# Autodesk Inventor assembly: 110033226_iam_10_角落碉堡
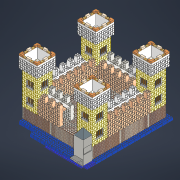
[picture p0: Inventor's stored thumbnail of the model, 180x180]
Saved by Autodesk Inventor 2022 (Build 260153000, 153)
## iProperties
Created: 2022-06-28
Part Number: 110033226_iam_10_角落碉堡
Document SubType Name: Assembly
Designer: User
Author: User
## Documents named in this file (8)
- D:\D-disk\pomelo\大一\下學期\機械設計製圖\1100332260_LEGOproj_沒有公主城堡\110033226_iam_10_角落碉堡.iam
- D:\D-disk\pomelo\大一\下學期\機械設計製圖\1100332260_LEGOproj_沒有公主城堡\110033226_ipt_43_角落碉堡基座.ipt
- D:\D-disk\pomelo\大一\下學期\機械設計製圖\1100332260_LEGOproj_沒有公主城堡\110033226_ipt_04_小河.ipt
- D:\D-disk\pomelo\大一\下學期\機械設計製圖\1100332260_LEGOproj_沒有公主城堡\110033226_iam_06_城堡四角塔.iam
- D:\D-disk\pomelo\大一\下學期\機械設計製圖\1100332260_LEGOproj_沒有公主城堡\110033226_ipt_34_中心城堡圍牆.ipt
- D:\D-disk\pomelo\大一\下學期\機械設計製圖\1100332260_LEGOproj_沒有公主城堡\110033226_ipt_24_直條(3x1).ipt
- D:\D-disk\pomelo\大一\下學期\機械設計製圖\1100332260_LEGOproj_沒有公主城堡\110033226_ipt_46_水中房子.ipt
- D:\D-disk\pomelo\大一\下學期\機械設計製圖\1100332260_LEGOproj_沒有公主城堡\110033226_ipt_37_小河方塊.ipt
## Components (310 placed, 7 different names)
1. 110033226_ipt_34_中心城堡圍牆:39 — 貼合:27, 貼合:28, 貼合:29, 貼合:38
2. 110033226_ipt_46_水中房子:1 — 貼合:39, 貼合:40, 貼合:41, 貼合:45, 貼合:46, 貼合:48, 貼合:50
3. 110033226_ipt_43_角落碉堡基座:1 — 貼合:1, 貼合:2, 貼合:3, 貼合:4, 貼合:5, 貼合:6, 貼合:7, 貼合:8, 貼合:9, 貼合:11, 貼合:39
4. 110033226_ipt_43_角落碉堡基座:2
5. 110033226_ipt_43_角落碉堡基座:3
6. 110033226_ipt_43_角落碉堡基座:4
7. 110033226_ipt_43_角落碉堡基座:5 — 貼合:40
8. 110033226_ipt_43_角落碉堡基座:6
9. 110033226_ipt_43_角落碉堡基座:7
10. 110033226_ipt_43_角落碉堡基座:8
11. 110033226_ipt_43_角落碉堡基座:9
12. 110033226_ipt_43_角落碉堡基座:10
13. 110033226_ipt_43_角落碉堡基座:11
14. 110033226_ipt_43_角落碉堡基座:12
15. 110033226_ipt_43_角落碉堡基座:13
16. 110033226_ipt_43_角落碉堡基座:14
17. 110033226_ipt_43_角落碉堡基座:15 — 貼合:12, 貼合:13, 貼合:14, 貼合:15, 貼合:16, 貼合:17, 貼合:18, 貼合:19, 貼合:21, 貼合:22, 貼合:23, 貼合:24, 貼合:25, 貼合:26, 貼合:27, 貼合:28, 貼合:29, 貼合:30, 貼合:31, 貼合:32, 貼合:33, 貼合:34, 貼合:35, 貼合:36, 貼合:37
18. 110033226_ipt_04_小河:4 — 貼合:7, 貼合:8, 貼合:9, 貼合:41, 貼合:42, 貼合:43, 貼合:44
19. 110033226_ipt_04_小河:5
20. 110033226_ipt_04_小河:6
21. 110033226_ipt_04_小河:7
22. 110033226_ipt_04_小河:8
23. 110033226_ipt_04_小河:9
24. 110033226_ipt_04_小河:10
25. 110033226_ipt_04_小河:11
26. 110033226_ipt_04_小河:12
27. 110033226_ipt_04_小河:13
28. 110033226_ipt_04_小河:14
29. 110033226_ipt_04_小河:15
30. 110033226_ipt_04_小河:16
31. 110033226_ipt_04_小河:17
32. 110033226_ipt_04_小河:18
33. 110033226_ipt_04_小河:19
34. 110033226_ipt_04_小河:20
35. 110033226_ipt_04_小河:21
36. 110033226_ipt_04_小河:22
37. 110033226_ipt_04_小河:23
38. 110033226_ipt_04_小河:24
39. 110033226_ipt_04_小河:25
40. 110033226_ipt_04_小河:26
41. 110033226_ipt_04_小河:27
42. 110033226_ipt_04_小河:28
43. 110033226_ipt_04_小河:29
44. 110033226_ipt_04_小河:30
45. 110033226_ipt_04_小河:31
46. 110033226_ipt_04_小河:32
47. 110033226_ipt_04_小河:33
48. 110033226_ipt_04_小河:34
49. 110033226_ipt_04_小河:35
50. 110033226_ipt_04_小河:36
51. 110033226_ipt_04_小河:37
52. 110033226_ipt_04_小河:38
53. 110033226_ipt_04_小河:39
54. 110033226_ipt_04_小河:40
55. 110033226_ipt_04_小河:41
56. 110033226_ipt_04_小河:42
57. 110033226_ipt_04_小河:43 — 對稱:1, 貼合:10
58. 110033226_ipt_04_小河:44
59. 110033226_ipt_04_小河:45
60. 110033226_ipt_04_小河:3 — 對稱:1, 貼合:10, 貼合:11
61. 110033226_ipt_04_小河:46
62. 110033226_ipt_04_小河:47
63. 110033226_ipt_04_小河:48
64. 110033226_ipt_04_小河:49
65. 110033226_ipt_04_小河:50
66. 110033226_ipt_04_小河:51
67. 110033226_ipt_04_小河:52
68. 110033226_ipt_04_小河:53
69. 110033226_ipt_04_小河:54
70. 110033226_ipt_04_小河:55
71. 110033226_ipt_04_小河:56
72. 110033226_ipt_04_小河:57
73. 110033226_ipt_04_小河:58
74. 110033226_ipt_04_小河:59
75. 110033226_ipt_04_小河:60
76. 110033226_ipt_04_小河:61
77. 110033226_ipt_04_小河:62
78. 110033226_ipt_04_小河:63
79. 110033226_ipt_04_小河:64
80. 110033226_ipt_04_小河:65
81. 110033226_ipt_04_小河:66
82. 110033226_ipt_04_小河:67
83. 110033226_ipt_04_小河:68
84. 110033226_ipt_04_小河:69
85. 110033226_ipt_04_小河:70
86. 110033226_ipt_04_小河:71
87. 110033226_ipt_04_小河:72
88. 110033226_ipt_04_小河:73
89. 110033226_ipt_04_小河:74
90. 110033226_ipt_04_小河:75
91. 110033226_ipt_04_小河:76
92. 110033226_ipt_04_小河:77
93. 110033226_ipt_04_小河:78
94. 110033226_ipt_04_小河:79
95. 110033226_ipt_04_小河:80
96. 110033226_ipt_04_小河:81
97. 110033226_ipt_04_小河:82
98. 110033226_ipt_04_小河:83
99. 110033226_iam_06_城堡四角塔:1 [sub-assembly] — 貼合:12, 貼合:13, 貼合:14
100. 110033226_iam_06_城堡四角塔:2 [sub-assembly]
101. 110033226_iam_06_城堡四角塔:3 [sub-assembly]
102. 110033226_iam_06_城堡四角塔:4 [sub-assembly]
103. 110033226_ipt_34_中心城堡圍牆:3 — 貼合:18, 貼合:19, 貼合:20
104. 110033226_ipt_34_中心城堡圍牆:1 — 貼合:15, 貼合:16, 貼合:17, 貼合:20
105. 110033226_ipt_34_中心城堡圍牆:5
106. 110033226_ipt_34_中心城堡圍牆:6
107. 110033226_ipt_34_中心城堡圍牆:7
108. 110033226_ipt_34_中心城堡圍牆:8
109. 110033226_ipt_34_中心城堡圍牆:9
110. 110033226_ipt_34_中心城堡圍牆:10
111. 110033226_ipt_34_中心城堡圍牆:11
112. 110033226_ipt_34_中心城堡圍牆:12
113. 110033226_ipt_34_中心城堡圍牆:13
114. 110033226_ipt_34_中心城堡圍牆:14
115. 110033226_ipt_34_中心城堡圍牆:15
116. 110033226_ipt_34_中心城堡圍牆:16
117. 110033226_ipt_34_中心城堡圍牆:17
118. 110033226_ipt_34_中心城堡圍牆:18
119. 110033226_ipt_34_中心城堡圍牆:19
120. 110033226_ipt_34_中心城堡圍牆:20
121. 110033226_ipt_34_中心城堡圍牆:21
122. 110033226_ipt_34_中心城堡圍牆:22
123. 110033226_ipt_34_中心城堡圍牆:23
124. 110033226_ipt_34_中心城堡圍牆:24
125. 110033226_ipt_34_中心城堡圍牆:25
126. 110033226_ipt_34_中心城堡圍牆:26
127. 110033226_ipt_34_中心城堡圍牆:28 — 貼合:25, 齊平:1, 貼合:26
128. 110033226_ipt_34_中心城堡圍牆:27 — 貼合:21, 貼合:22, 貼合:23, 貼合:24, 齊平:1
129. 110033226_ipt_34_中心城堡圍牆:29
130. 110033226_ipt_34_中心城堡圍牆:30
131. 110033226_ipt_34_中心城堡圍牆:31
132. 110033226_ipt_34_中心城堡圍牆:32
133. 110033226_ipt_34_中心城堡圍牆:33
134. 110033226_ipt_34_中心城堡圍牆:34
135. 110033226_ipt_34_中心城堡圍牆:35
136. 110033226_ipt_34_中心城堡圍牆:36
137. 110033226_ipt_34_中心城堡圍牆:37
138. 110033226_ipt_34_中心城堡圍牆:38
139. 110033226_ipt_34_中心城堡圍牆:41 — 貼合:33, 貼合:34, 貼合:35
140. 110033226_ipt_34_中心城堡圍牆:40 — 貼合:30, 貼合:31, 貼合:32
141. 110033226_ipt_34_中心城堡圍牆:42
142. 110033226_ipt_34_中心城堡圍牆:43
143. 110033226_ipt_37_小河方塊:21 — 貼合:45, 貼合:46, 貼合:47
144. 110033226_ipt_37_小河方塊:22
145. 110033226_ipt_37_小河方塊:23
146. 110033226_ipt_37_小河方塊:24
147. 110033226_ipt_37_小河方塊:25
148. 110033226_ipt_37_小河方塊:26 — 貼合:49
149. 110033226_ipt_37_小河方塊:27
150. 110033226_ipt_37_小河方塊:28
151. 110033226_ipt_37_小河方塊:29
152. 110033226_ipt_37_小河方塊:30
153. 110033226_ipt_37_小河方塊:31
154. 110033226_ipt_37_小河方塊:32
155. 110033226_ipt_37_小河方塊:33
156. 110033226_ipt_37_小河方塊:34
157. 110033226_ipt_37_小河方塊:35
158. 110033226_ipt_37_小河方塊:36
159. 110033226_ipt_37_小河方塊:37
160. 110033226_ipt_37_小河方塊:38
161. 110033226_ipt_37_小河方塊:39
162. 110033226_ipt_37_小河方塊:40
163. 110033226_ipt_24_直條(3x1):1 — 貼合:36, 貼合:37, 貼合:38
164. 110033226_ipt_24_直條(3x1):2
165. 110033226_ipt_24_直條(3x1):3
166. 110033226_ipt_24_直條(3x1):4
167. 110033226_ipt_24_直條(3x1):5
168. 110033226_ipt_24_直條(3x1):6
169. 110033226_ipt_24_直條(3x1):7
170. 110033226_ipt_24_直條(3x1):8
171. 110033226_ipt_24_直條(3x1):9
172. 110033226_ipt_24_直條(3x1):10
173. 110033226_ipt_24_直條(3x1):11
174. 110033226_ipt_24_直條(3x1):12
175. 110033226_ipt_37_小河方塊:1 — 貼合:42, 貼合:43, 貼合:44
176. 110033226_ipt_37_小河方塊:2
177. 110033226_ipt_37_小河方塊:3
178. 110033226_ipt_37_小河方塊:4
179. 110033226_ipt_37_小河方塊:5
180. 110033226_ipt_37_小河方塊:6
181. 110033226_ipt_37_小河方塊:7
182. 110033226_ipt_37_小河方塊:8
183. 110033226_ipt_37_小河方塊:9
184. 110033226_ipt_37_小河方塊:10 — 貼合:47
185. 110033226_ipt_37_小河方塊:11
186. 110033226_ipt_37_小河方塊:12
187. 110033226_ipt_37_小河方塊:13
188. 110033226_ipt_37_小河方塊:14
189. 110033226_ipt_37_小河方塊:15
190. 110033226_ipt_37_小河方塊:16
191. 110033226_ipt_37_小河方塊:17
192. 110033226_ipt_37_小河方塊:18
193. 110033226_ipt_37_小河方塊:19
194. 110033226_ipt_37_小河方塊:20
195. 110033226_ipt_04_小河:88 — 貼合:48, 貼合:49, 貼合:50
196. 110033226_ipt_04_小河:89
197. 110033226_ipt_04_小河:90
198. 110033226_ipt_04_小河:91
199. 110033226_ipt_04_小河:92
200. 110033226_ipt_04_小河:93
201. 110033226_ipt_04_小河:94
202. 110033226_ipt_04_小河:95
203. 110033226_ipt_04_小河:96
204. 110033226_ipt_04_小河:97
205. 110033226_ipt_04_小河:98
206. 110033226_ipt_04_小河:99
207. 110033226_ipt_04_小河:100
208. 110033226_ipt_04_小河:101
209. 110033226_ipt_04_小河:102
210. 110033226_ipt_04_小河:103
211. 110033226_ipt_04_小河:104
212. 110033226_ipt_04_小河:105
213. 110033226_ipt_04_小河:106
214. 110033226_ipt_04_小河:107
215. 110033226_ipt_04_小河:108
216. 110033226_ipt_04_小河:109
217. 110033226_ipt_04_小河:110
218. 110033226_ipt_04_小河:111
219. 110033226_ipt_04_小河:1 — 貼合:4, 貼合:5, 貼合:6
220. 110033226_ipt_04_小河:84
221. 110033226_ipt_04_小河:85
222. 110033226_ipt_04_小河:86
223. 110033226_ipt_04_小河:87
224. 110033226_ipt_04_小河:112
225. 110033226_ipt_04_小河:113
226. 110033226_ipt_04_小河:114
227. 110033226_ipt_04_小河:115
228. 110033226_ipt_04_小河:116
229. 110033226_ipt_04_小河:117
230. 110033226_ipt_04_小河:118
231. 110033226_ipt_04_小河:119
232. 110033226_ipt_04_小河:120
233. 110033226_ipt_04_小河:121
234. 110033226_ipt_04_小河:122
235. 110033226_ipt_04_小河:123
236. 110033226_ipt_04_小河:124
237. 110033226_ipt_04_小河:125
238. 110033226_ipt_04_小河:126
239. 110033226_ipt_04_小河:127
240. 110033226_ipt_04_小河:128
241. 110033226_ipt_04_小河:129
242. 110033226_ipt_04_小河:130
243. 110033226_ipt_04_小河:131
244. 110033226_ipt_04_小河:132
245. 110033226_ipt_04_小河:133
246. 110033226_ipt_04_小河:134
247. 110033226_ipt_04_小河:135
248. 110033226_ipt_04_小河:136
249. 110033226_ipt_04_小河:137
250. 110033226_ipt_04_小河:138
251. 110033226_ipt_04_小河:139
252. 110033226_ipt_04_小河:140
253. 110033226_ipt_04_小河:141
254. 110033226_ipt_04_小河:142
255. 110033226_ipt_04_小河:143
256. 110033226_ipt_04_小河:144
257. 110033226_ipt_04_小河:145
258. 110033226_ipt_04_小河:146
259. 110033226_ipt_04_小河:147
260. 110033226_ipt_04_小河:148
261. 110033226_ipt_04_小河:149
262. 110033226_ipt_04_小河:150
263. 110033226_ipt_04_小河:151
264. 110033226_ipt_04_小河:152
265. 110033226_ipt_04_小河:153
266. 110033226_ipt_04_小河:154
267. 110033226_ipt_04_小河:155
268. 110033226_ipt_04_小河:156
269. 110033226_ipt_04_小河:157
270. 110033226_ipt_04_小河:158
271. 110033226_ipt_04_小河:159
272. 110033226_ipt_04_小河:160
273. 110033226_ipt_04_小河:161
274. 110033226_ipt_04_小河:162
275. 110033226_ipt_04_小河:163
276. 110033226_ipt_04_小河:164
277. 110033226_ipt_04_小河:165
278. 110033226_ipt_04_小河:166
279. 110033226_ipt_04_小河:167
280. 110033226_ipt_04_小河:168
281. 110033226_ipt_04_小河:169
282. 110033226_ipt_04_小河:170
283. 110033226_ipt_04_小河:171
284. 110033226_ipt_04_小河:172
285. 110033226_ipt_04_小河:173
286. 110033226_ipt_04_小河:174
287. 110033226_ipt_04_小河:175
288. 110033226_ipt_04_小河:176
289. 110033226_ipt_04_小河:177
290. 110033226_ipt_04_小河:178
291. 110033226_ipt_04_小河:179
292. 110033226_ipt_04_小河:180
293. 110033226_ipt_04_小河:181
294. 110033226_ipt_04_小河:182
295. 110033226_ipt_04_小河:183
296. 110033226_ipt_04_小河:184
297. 110033226_ipt_04_小河:185
298. 110033226_ipt_04_小河:186
299. 110033226_ipt_04_小河:187
300. 110033226_ipt_04_小河:188
301. 110033226_ipt_04_小河:189
302. 110033226_ipt_04_小河:190
303. 110033226_ipt_04_小河:191
304. 110033226_ipt_04_小河:192
305. 110033226_ipt_04_小河:193
306. 110033226_ipt_04_小河:194
307. 110033226_ipt_04_小河:195
308. 110033226_ipt_04_小河:196
309. 110033226_ipt_04_小河:197
310. 110033226_ipt_04_小河:198
## Component patterns: (15 elements, first: 110033226_ipt_43_角落碉堡基座:1), (42 elements, first: 110033226_ipt_04_小河:4), (39 elements, first: 110033226_ipt_04_小河:3), (4 elements, first: 110033226_iam_06_城堡四角塔:1), (12 elements, first: 110033226_ipt_34_中心城堡圍牆:3 + 110033226_ipt_34_中心城堡圍牆:1), (6 elements, first: 110033226_ipt_34_中心城堡圍牆:28 + 110033226_ipt_34_中心城堡圍牆:27), (2 elements, first: 110033226_ipt_34_中心城堡圍牆:41 + 110033226_ipt_34_中心城堡圍牆:40), (3 elements), (2 elements), (20 elements, first: 110033226_ipt_37_小河方塊:21), (4 elements), (4 elements, first: 110033226_ipt_24_直條(3x1):1), 元件陣列 11:2 (4 elements), 元件陣列 11:3 (4 elements), (10 elements, first: 110033226_ipt_37_小河方塊:1), 元件陣列 13:2 (10 elements), (24 elements, first: 110033226_ipt_04_小河:88), (5 elements, first: 110033226_ipt_04_小河:1), 元件陣列 16:2 (24 elements), 元件陣列 4:2 (5 elements), 元件陣列 16:3 (24 elements), 元件陣列 4:3 (5 elements), 元件陣列 16:4 (24 elements), 元件陣列 4:4 (5 elements)
## Relationships (52: Mate 50, Symmetry 1, Flush 1)
- 貼合:1 [Mate]: 110033226_ipt_43_角落碉堡基座:1
- 貼合:2 [Mate]: 110033226_ipt_43_角落碉堡基座:1
- 貼合:3 [Mate]: 110033226_ipt_43_角落碉堡基座:1
- 貼合:4 [Mate]: 110033226_ipt_43_角落碉堡基座:1 ↔ 110033226_ipt_04_小河:1
- 貼合:5 [Mate]: 110033226_ipt_43_角落碉堡基座:1 ↔ 110033226_ipt_04_小河:1
- 貼合:6 [Mate]: 110033226_ipt_43_角落碉堡基座:1 ↔ 110033226_ipt_04_小河:1
- 貼合:7 [Mate]: 110033226_ipt_43_角落碉堡基座:1 ↔ 110033226_ipt_04_小河:4
- 貼合:8 [Mate]: 110033226_ipt_43_角落碉堡基座:1 ↔ 110033226_ipt_04_小河:4
- 貼合:9 [Mate]: 110033226_ipt_43_角落碉堡基座:1 ↔ 110033226_ipt_04_小河:4
- 對稱:1 [Symmetry]: 110033226_ipt_04_小河:43 ↔ 110033226_ipt_04_小河:3
- 貼合:10 [Mate]: 110033226_ipt_04_小河:43 ↔ 110033226_ipt_04_小河:3
- 貼合:11 [Mate]: 110033226_ipt_43_角落碉堡基座:1 ↔ 110033226_ipt_04_小河:3
- 貼合:12 [Mate]: 110033226_ipt_43_角落碉堡基座:15 ↔ 110033226_iam_06_城堡四角塔:1
- 貼合:13 [Mate]: 110033226_ipt_43_角落碉堡基座:15 ↔ 110033226_iam_06_城堡四角塔:1
- 貼合:14 [Mate]: 110033226_ipt_43_角落碉堡基座:15 ↔ 110033226_iam_06_城堡四角塔:1
- 貼合:15 [Mate]: 110033226_ipt_43_角落碉堡基座:15 ↔ 110033226_ipt_34_中心城堡圍牆:1
- 貼合:16 [Mate]: 110033226_ipt_43_角落碉堡基座:15 ↔ 110033226_ipt_34_中心城堡圍牆:1
- 貼合:17 [Mate]: 110033226_ipt_43_角落碉堡基座:15 ↔ 110033226_ipt_34_中心城堡圍牆:1
- 貼合:18 [Mate]: 110033226_ipt_43_角落碉堡基座:15 ↔ 110033226_ipt_34_中心城堡圍牆:3
- 貼合:19 [Mate]: 110033226_ipt_43_角落碉堡基座:15 ↔ 110033226_ipt_34_中心城堡圍牆:3
- 貼合:20 [Mate]: 110033226_ipt_34_中心城堡圍牆:3 ↔ 110033226_ipt_34_中心城堡圍牆:1
- 貼合:21 [Mate]: 110033226_ipt_43_角落碉堡基座:15 ↔ 110033226_ipt_34_中心城堡圍牆:27
- 貼合:22 [Mate]: 110033226_ipt_43_角落碉堡基座:15 ↔ 110033226_ipt_34_中心城堡圍牆:27
- 貼合:23 [Mate]: 110033226_ipt_43_角落碉堡基座:15 ↔ 110033226_ipt_34_中心城堡圍牆:27
- 貼合:24 [Mate]: 110033226_ipt_43_角落碉堡基座:15 ↔ 110033226_ipt_34_中心城堡圍牆:27
- 貼合:25 [Mate]: 110033226_ipt_43_角落碉堡基座:15 ↔ 110033226_ipt_34_中心城堡圍牆:28
- 齊平:1 [Flush]: 110033226_ipt_34_中心城堡圍牆:28 ↔ 110033226_ipt_34_中心城堡圍牆:27
- 貼合:26 [Mate]: 110033226_ipt_43_角落碉堡基座:15 ↔ 110033226_ipt_34_中心城堡圍牆:28
- 貼合:27 [Mate]: 110033226_ipt_34_中心城堡圍牆:39 ↔ 110033226_ipt_43_角落碉堡基座:15
- 貼合:28 [Mate]: 110033226_ipt_34_中心城堡圍牆:39 ↔ 110033226_ipt_43_角落碉堡基座:15
- 貼合:29 [Mate]: 110033226_ipt_34_中心城堡圍牆:39 ↔ 110033226_ipt_43_角落碉堡基座:15
- 貼合:30 [Mate]: 110033226_ipt_43_角落碉堡基座:15 ↔ 110033226_ipt_34_中心城堡圍牆:40
- 貼合:31 [Mate]: 110033226_ipt_43_角落碉堡基座:15 ↔ 110033226_ipt_34_中心城堡圍牆:40
- 貼合:32 [Mate]: 110033226_ipt_43_角落碉堡基座:15 ↔ 110033226_ipt_34_中心城堡圍牆:40
- 貼合:33 [Mate]: 110033226_ipt_43_角落碉堡基座:15 ↔ 110033226_ipt_34_中心城堡圍牆:41
- 貼合:34 [Mate]: 110033226_ipt_43_角落碉堡基座:15 ↔ 110033226_ipt_34_中心城堡圍牆:41
- 貼合:35 [Mate]: 110033226_ipt_43_角落碉堡基座:15 ↔ 110033226_ipt_34_中心城堡圍牆:41
- 貼合:36 [Mate]: 110033226_ipt_43_角落碉堡基座:15 ↔ 110033226_ipt_24_直條(3x1):1
- 貼合:37 [Mate]: 110033226_ipt_43_角落碉堡基座:15 ↔ 110033226_ipt_24_直條(3x1):1
- 貼合:38 [Mate]: 110033226_ipt_34_中心城堡圍牆:39 ↔ 110033226_ipt_24_直條(3x1):1
- 貼合:39 [Mate]: 110033226_ipt_46_水中房子:1 ↔ 110033226_ipt_43_角落碉堡基座:1
- 貼合:40 [Mate]: 110033226_ipt_46_水中房子:1 ↔ 110033226_ipt_43_角落碉堡基座:5
- 貼合:41 [Mate]: 110033226_ipt_46_水中房子:1 ↔ 110033226_ipt_04_小河:4
- 貼合:42 [Mate]: 110033226_ipt_04_小河:4 ↔ 110033226_ipt_37_小河方塊:1
- 貼合:43 [Mate]: 110033226_ipt_04_小河:4 ↔ 110033226_ipt_37_小河方塊:1
- 貼合:44 [Mate]: 110033226_ipt_04_小河:4 ↔ 110033226_ipt_37_小河方塊:1
- 貼合:45 [Mate]: 110033226_ipt_46_水中房子:1 ↔ 110033226_ipt_37_小河方塊:21
- 貼合:46 [Mate]: 110033226_ipt_46_水中房子:1 ↔ 110033226_ipt_37_小河方塊:21
- 貼合:47 [Mate]: 110033226_ipt_37_小河方塊:21 ↔ 110033226_ipt_37_小河方塊:10
- 貼合:48 [Mate]: 110033226_ipt_46_水中房子:1 ↔ 110033226_ipt_04_小河:88
- 貼合:49 [Mate]: 110033226_ipt_37_小河方塊:26 ↔ 110033226_ipt_04_小河:88
- 貼合:50 [Mate]: 110033226_ipt_46_水中房子:1 ↔ 110033226_ipt_04_小河:88
